# Autodesk Inventor assembly: 4198
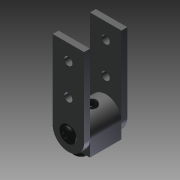
[picture p0: Inventor's stored thumbnail of the model, 180x180]
Saved by Autodesk Inventor 2016 (Build 200138000, 138)
## iProperties
Category: PARTsolutions
Company: 8020
Created: 2016-04-17
Part Number: 4198
Catalog Web Link: www.cadenas.de
Description: 4198-Standard Pivot Nub Assemblies - 10 Series - 90 deg 3 Inch Arm Pivot
Vendor: 8020
Document SubType Name: Assembly
Designer: psAdmin
Manufacturer: 8020
PSOL_IDENT_0: {$CADENAS_DATA\23d-libs\8020\inch\joining_plates\4198_asmtab.prj},144 {VTYP=3D},{STYP=ASSTAB},{NB=41
PSOL_IDENT_1: 98},{LINA=4198},{NN=4198},{DATE=22.08.2012},{GEOMDATE=16.01.2012},{VERSION=},{LINEID=10},{LINESUBID=
PSOL_IDENT_2: -1},{WBVAR=}  {NB=4198},{LINA=4198},{KT=DUMMY},{PN=4198},{DPN=4188},{PA=4196},{L=0.50000000},{IMH1=1
PSOL_IDENT_3: /4-20},{PPATH=4198_asmtpl.prj},{A=1.000},{B=3.000},{C=0.500},{D=1.000},{DIA=0.257},{E=0.443},{F=1.00
PSOL_IDENT_4: 0},{G=0.094},{H=0.500},{I=1.376},{T=0.188},{W=.190},{MHIP=1/4-20 x 1 Inch SHCS and Economy T-Nut },{
PSOL_IDENT_5: MHIA=1/4-20 x 1/2 Inch FBHSCS}
NN: 4198
NT: Standard Pivot Nub Assemblies - 10 Series - 90 deg 3 Inch Arm Pivot
NB: 4198
NBSYN: $PN.
LINA: 4198
PN: 4198
A: 1.000
B: 3.000
C: 0.500
D: 1.000
DIA: 0.257
E: 0.443
F: 1.000
G: 0.094
H: 0.500
I: 1.376
T: 0.188
W: .190
SUPPLIER: 8020
ARTICLENO: 4198
BOMINFO: 4198
CREATOR: CADENAS GmbH
Title: 4198
Author: Cadenas PARTsolutions
Comments: Standard Pivot Nub Assemblies - 10 Series - 90 deg 3 Inch Arm Pivot
## Documents named in this file (6)
- C:\Users\Haden\Desktop\Cad-Model\Monitor\Structural Pivot-8020-4198\Structural Pivot-8020-4198.iam
- C:\Users\Haden\Desktop\Cad-Model\Monitor\Structural Pivot-8020-4198\4188_n.ipt
- C:\Users\Haden\Desktop\Cad-Model\Monitor\Structural Pivot-8020-4198\4196.ipt
- C:\Users\Haden\Desktop\Cad-Model\Monitor\Structural Pivot-8020-4198\3342.ipt
- C:\Users\Haden\Desktop\Cad-Model\Monitor\Structural Pivot-8020-4198\3071.ipt
- C:\Users\Haden\Desktop\Cad-Model\Monitor\Structural Pivot-8020-4198\3382.ipt
## Components (7 placed, 5 different names)
1. 4188_n:1 — Insert:1, Insert:2, Angle:1
2. 4196:1 — Insert:1, Flush:1
3. 3342:1
4. 3071:1
5. 3382:1
6. 4196:2 — Insert:2, Flush:1, Angle:1
7. 3342:2
## Relationships (4: Insert 2, Flush 1, Angle 1)
- Insert:1: 4188_n:1 ↔ 4196:1
- Insert:2: 4188_n:1 ↔ 4196:2
- Flush:1: 4196:1 ↔ 4196:2
- Angle:1 (180 deg): 4188_n:1 ↔ 4196:2
